# Autodesk Inventor assembly: Assembly2
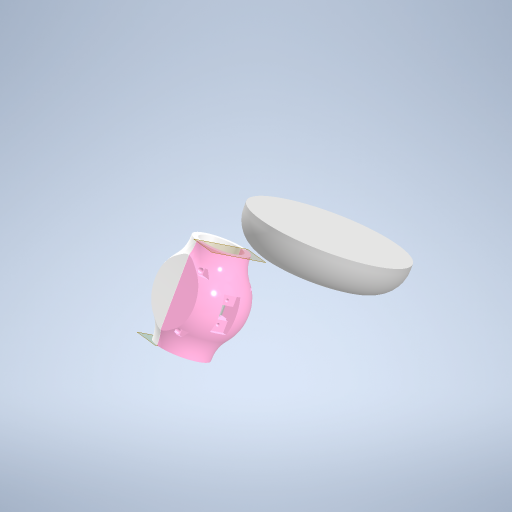
[picture p0: Inventor's stored thumbnail of the model, 512x512]
Saved by Autodesk Inventor 2023 (Build 270158000, 158)
## iProperties
Created: 2022-11-07
Part Number: Assembly2
Document SubType Name: Assembly
Designer: RM206user
Author: RM206user
## Documents named in this file (3)
- C:\Users\RM206user\Desktop\cansat\tanekonsat2022_runback\machinary\assenbly\Assembly2.iam
- C:\Users\RM206user\Desktop\cansat\tanekonsat2022_runback\machinary\assenbly\Assembly1.iam
- C:\Users\RM206user\Desktop\cansat\tanekonsat2022_runback\machinary\parts\tire\wheel 2.ipt
## Components (2 placed, 2 different names)
1. Assembly1:1 [sub-assembly] — メイト:1, メイト:5, メイト:6
2. wheel 2:1 — メイト:1, メイト:2, メイト:3, メイト:4, メイト:5, メイト:6
## Relationships (6: Mate 6)
- メイト:1 [Mate] (-10 mm): Assembly1:1 ↔ wheel 2:1
- メイト:2 [Mate]: wheel 2:1
- メイト:3 [Mate]: wheel 2:1
- メイト:4 [Mate]: wheel 2:1
- メイト:5 [Mate]: Assembly1:1 ↔ wheel 2:1
- メイト:6 [Mate]: Assembly1:1 ↔ wheel 2:1
